# Autodesk Inventor assembly: Temp_Assembly1
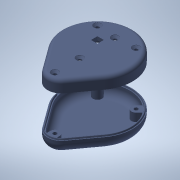
[picture p0: Inventor's stored thumbnail of the model, 180x180]
Saved by Autodesk Inventor 2020 (Build 240168000, 168)
## iProperties
Created: 2020-12-01
Part Number: Temp_Assembly1
Document SubType Name: Assembly
Designer: sandr
Author: sandr
## Documents named in this file (3)
- C:\Users\sandr\OneDrive\Formacion\Universidad\2020-2\Fundamentos de biodiseño\Modelado\Case v3\Temp_Assembly1.iam
- C:\Users\sandr\OneDrive\Formacion\Universidad\2020-2\Fundamentos de biodiseño\Modelado\Case v3\front_temp.ipt
- C:\Users\sandr\OneDrive\Formacion\Universidad\2020-2\Fundamentos de biodiseño\Modelado\Case v3\back_temp.ipt
## Components (2 placed, 2 different names)
1. front_temp:1 — Mate:1, Mate:2
2. back_temp:1 — Mate:1, Mate:2
## Relationships (2: Mate 2)
- Mate:1: front_temp:1 ↔ back_temp:1
- Mate:2: front_temp:1 ↔ back_temp:1
